# Autodesk Inventor assembly: ASM_Vial_and_Header
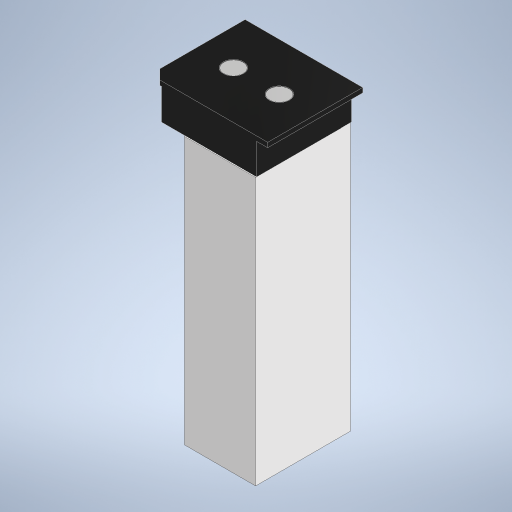
[picture p0: Inventor's stored thumbnail of the model, 512x512]
Saved by Autodesk Inventor 2024 (Build 280153000, 153)
## iProperties
Created: 2024-04-23
Part Number: ASM_Vial_and_Header
Document SubType Name: Assembly
Designer: jamha
Author: jamha
## Documents named in this file (4)
- C:\Users\jamha\OneDrive - The University of Texas at Dallas\SD - TEAM 1830\CAD\James\Sample Tray Assembly V2\ASM_Vial_and_Header.iam
- C:\Users\jamha\OneDrive - The University of Texas at Dallas\SD - TEAM 1830\CAD\James\Sample Tray Assembly V2\Custom Made Vial.ipt
- C:\Users\jamha\OneDrive - The University of Texas at Dallas\SD - TEAM 1830\CAD\James\Sample Tray Assembly V2\Header Final Design.ipt
- C:\Users\jamha\OneDrive - The University of Texas at Dallas\SD - TEAM 1830\CAD\James\Sample Tray Assembly V2\Neodynium Magnet\5862K103_Neodymium Magnet\5862K103_Neodymium Magnet.ipt
## Components (4 placed, 3 different names)
1. Custom Made Vial:1 — Mate:1, Angle:1, Mate:6
2. Header Final Design:1 — Mate:1, Angle:1, Mate:2, Mate:3, Mate:4, Mate:5, Mate:6
3. 5862K103_Neodymium Magnet:1 — Mate:2, Mate:3
4. 5862K103_Neodymium Magnet:2 — Mate:4, Mate:5
## Relationships (7: Mate 6, Angle 1)
- Mate:1: Custom Made Vial:1 ↔ Header Final Design:1
- Angle:1 (0 deg): Custom Made Vial:1 ↔ Header Final Design:1
- Mate:2: Header Final Design:1 ↔ 5862K103_Neodymium Magnet:1
- Mate:3: Header Final Design:1 ↔ 5862K103_Neodymium Magnet:1
- Mate:4: Header Final Design:1 ↔ 5862K103_Neodymium Magnet:2
- Mate:5: Header Final Design:1 ↔ 5862K103_Neodymium Magnet:2
- Mate:6: Custom Made Vial:1 ↔ Header Final Design:1
